# Autodesk Inventor assembly: print008_Guss_mit_Einsatz
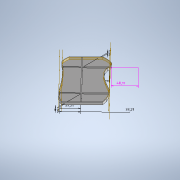
[picture p0: Inventor's stored thumbnail of the model, 180x180]
Saved by Autodesk Inventor 2020.3 (Build 243373000, 373)
## iProperties
Created: 2020-06-25
Part Number: print008_Guss_mit_Einsatz
Document SubType Name: Assembly
Designer: Mara
Mass: 14.6297 g
Surface Area: 295.485 cm^2
Volume: 14.6297 cm^3
Density: 1 g/cm^3
Author: Mara
## Documents named in this file (3)
- C:\Users\Mara\Masterarbeit_CAD\print008_Guss_mit_Einsatz.iam
- C:\Users\Mara\Masterarbeit_CAD\print008_Grundform_Guss.ipt
- C:\Users\Mara\Masterarbeit_CAD\print008_Grundform_Guss_innen.ipt
## Components (2 placed, 2 different names)
1. print008_Grundform_Guss:1
2. print008_Grundform_Guss_innen:1 — Flush:1, Flush:2, Flush:3, Flush:4
## Relationships (4: Flush 4)
- Flush:1 (48.61 mm): print008_Grundform_Guss_innen:1
- Flush:2 (47.67 mm): print008_Grundform_Guss_innen:1
- Flush:3 (38.21 mm): print008_Grundform_Guss_innen:1
- Flush:4 (32.91 mm): print008_Grundform_Guss_innen:1
